# Autodesk Inventor assembly: armAssembaly
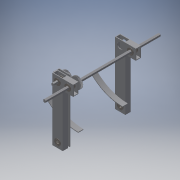
[picture p0: Inventor's stored thumbnail of the model, 180x180]
Saved by Autodesk Inventor 2016 (Build 200138000, 138)
## iProperties
Created: 2016-01-27
Part Number: armAssembaly
Document SubType Name: Assembly
Designer: 278648
Author: 278648
## Documents named in this file (11)
- \\Mac\Home\Downloads\robotwithshooterandaiming-2\1510-stronghold-CAD-master\pickeruperthingy\armAssembaly.iam
- \\Mac\Home\Downloads\robotwithshooterandaiming-2\1510-stronghold-CAD-master\pickeruperthingy\arm.ipt
- \\Mac\Home\Downloads\robotwithshooterandaiming-2\1510-stronghold-CAD-master\pickeruperthingy\217-3875-STEP-20140818.ipt
- \\Mac\Home\Downloads\robotwithshooterandaiming-2\1510-stronghold-CAD-master\pickeruperthingy\rod.ipt
- \\Mac\Home\Downloads\robotwithshooterandaiming-2\1510-stronghold-CAD-master\pickeruperthingy\rod2.ipt
- \\Mac\Home\Downloads\robotwithshooterandaiming-2\1510-stronghold-CAD-master\pickeruperthingy\217-2708.20121204.ipt
- \\Mac\Home\Downloads\robotwithshooterandaiming-2\1510-stronghold-CAD-master\pickeruperthingy\217-3488-STEP.ipt
- \\Mac\Home\Downloads\robotwithshooterandaiming-2\1510-stronghold-CAD-master\pickeruperthingy\Part13.ipt
- \\Mac\Home\Downloads\robotwithshooterandaiming-2\1510-stronghold-CAD-master\pickeruperthingy\chainguard.ipt
- \\Mac\Home\Downloads\robotwithshooterandaiming-2\1510-stronghold-CAD-master\pickeruperthingy\arm_new1.ipt
- \\Mac\Home\Downloads\robotwithshooterandaiming-2\1510-stronghold-CAD-master\pickeruperthingy\railholderleft.ipt
## Components (21 placed, 10 different names)
1. arm:1 — Mate:2, Mate:3, Mate:6, Mate:9, Mate:16, Mate:17, Mate:18, Mate:19, Mate:22, Mate:23, Mate:24, Mate:25, Mate:43, Mate:44, Mate:60, Flush:9, Flush:10, Mate:62, Flush:14, Mate:69, Flush:16
2. 217-3875-STEP-20140818:1 — Mate:2, Mate:3, Mate:10, Mate:11
3. 217-3875-STEP-20140818:2 — Mate:63, Mate:64, Mate:67, Mate:68
4. 217-3875-STEP-20140818:3 — Mate:52, Mate:65, Mate:66
5. 217-3875-STEP-20140818:4 — Mate:6, Mate:9, Mate:51
6. rod:1 — Mate:10, Mate:11, Mate:34, Mate:35, Mate:67, Mate:68, Flush:14
7. 217-3875-STEP-20140818:7 — Mate:18, Mate:19
8. 217-3875-STEP-20140818:8 — Mate:16, Mate:17
9. 217-3875-STEP-20140818:9 — Mate:22, Mate:23
10. 217-3875-STEP-20140818:12 — Mate:24, Mate:25, Mate:30, Mate:31
11. rod2:2 — Mate:30, Mate:31, Mate:32, Mate:33, Mate:56, Mate:57, Flush:12
12. 217-2708.20121204:1 — Mate:32, Mate:33, Mate:44, Flush:12
13. 217-2708.20121204:2 — Mate:34, Mate:35, Mate:43
14. 217-3488-STEP:1 — Flush:7, Mate:56, Mate:57, Mate:62
15. 217-3488-STEP:2 — Flush:7
16. Part13:1 — Mate:51, Mate:53, Flush:8, Flush:15
17. Part13:2 — Mate:52, Mate:53, Flush:8, Mate:61, Mate:70
18. chainguard:1 — Mate:60, Flush:9, Flush:10, Mate:61, Mate:71
19. arm_new1:1 — Mate:63, Mate:64, Mate:65, Mate:66, Flush:15, Mate:69, Flush:16, Mate:72
20. railholderleft:1 — Mate:70, Mate:71, Flush:17, Flush:18
21. railholderleft:2 — Flush:17, Flush:18, Mate:72
## Relationships (50: Mate 40, Flush 10)
- Mate:2: arm:1 ↔ 217-3875-STEP-20140818:1
- Mate:3: arm:1 ↔ 217-3875-STEP-20140818:1
- Mate:6: arm:1 ↔ 217-3875-STEP-20140818:4
- Mate:9: arm:1 ↔ 217-3875-STEP-20140818:4
- Mate:10: 217-3875-STEP-20140818:1 ↔ rod:1
- Mate:11: 217-3875-STEP-20140818:1 ↔ rod:1
- Mate:16: arm:1 ↔ 217-3875-STEP-20140818:8
- Mate:17: arm:1 ↔ 217-3875-STEP-20140818:8
- Mate:18: arm:1 ↔ 217-3875-STEP-20140818:7
- Mate:19: arm:1 ↔ 217-3875-STEP-20140818:7
- Mate:22: arm:1 ↔ 217-3875-STEP-20140818:9
- Mate:23: arm:1 ↔ 217-3875-STEP-20140818:9
- Mate:24: arm:1 ↔ 217-3875-STEP-20140818:12
- Mate:25: arm:1 ↔ 217-3875-STEP-20140818:12
- Mate:30: 217-3875-STEP-20140818:12 ↔ rod2:2
- Mate:31: 217-3875-STEP-20140818:12 ↔ rod2:2
- Mate:32: rod2:2 ↔ 217-2708.20121204:1
- Mate:33: rod2:2 ↔ 217-2708.20121204:1
- Mate:34: rod:1 ↔ 217-2708.20121204:2
- Mate:35: rod:1 ↔ 217-2708.20121204:2
- Mate:43 (12.7 mm): arm:1 ↔ 217-2708.20121204:2
- Mate:44 (12.7 mm): arm:1 ↔ 217-2708.20121204:1
- Flush:7: 217-3488-STEP:1 ↔ 217-3488-STEP:2
- Mate:51: 217-3875-STEP-20140818:4 ↔ Part13:1
- Mate:52: 217-3875-STEP-20140818:3 ↔ Part13:2
- Mate:53 (190.5 mm): Part13:1 ↔ Part13:2
- Flush:8: Part13:1 ↔ Part13:2
- Mate:56: rod2:2 ↔ 217-3488-STEP:1
- Mate:57: rod2:2 ↔ 217-3488-STEP:1
- Mate:60 (8.255 mm): arm:1 ↔ chainguard:1
- Flush:9: arm:1 ↔ chainguard:1
- Flush:10: arm:1 ↔ chainguard:1
- Mate:61 (13.335 mm): Part13:2 ↔ chainguard:1
- Mate:62 (3.175 mm): arm:1 ↔ 217-3488-STEP:1
- Flush:12 (-3.175 mm): rod2:2 ↔ 217-2708.20121204:1
- Mate:63: 217-3875-STEP-20140818:2 ↔ arm_new1:1
- Mate:64: 217-3875-STEP-20140818:2 ↔ arm_new1:1
- Mate:65: 217-3875-STEP-20140818:3 ↔ arm_new1:1
- Mate:66: 217-3875-STEP-20140818:3 ↔ arm_new1:1
- Mate:67: 217-3875-STEP-20140818:2 ↔ rod:1
- Mate:68: 217-3875-STEP-20140818:2 ↔ rod:1
- Flush:14 (-114.3 mm): arm:1 ↔ rod:1
- Flush:15 (25.4 mm): Part13:1 ↔ arm_new1:1
- Mate:69 (-330.2 mm): arm:1 ↔ arm_new1:1
- Flush:16: arm:1 ↔ arm_new1:1
- Mate:70: Part13:2 ↔ railholderleft:1
- Mate:71: chainguard:1 ↔ railholderleft:1
- Flush:17: railholderleft:1 ↔ railholderleft:2
- Flush:18: railholderleft:1 ↔ railholderleft:2
- Mate:72: arm_new1:1 ↔ railholderleft:2
